# Autodesk Inventor assembly: Vex Pulley 9 mm - 42T
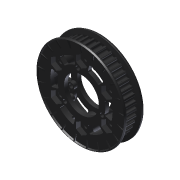
[picture p0: Inventor's stored thumbnail of the model, 180x180]
Saved by Autodesk Inventor 2013 (Build 170138000, 138)
## iProperties
Created: 2013-12-20
Part Number: Vex Pulley 9 mm - 42T
Document SubType Name: Assembly
Designer: Nemo
Author: Nemo
## Documents named in this file (2)
- H:\Nemo\Documents\Robotics\COTS Parts\Pulleys - Vex\Vex Pulley 9 mm - 42T.iam
- H:\Nemo\Documents\Robotics\COTS Parts\Pulleys - Vex\Components\Vex VersaPulley 42T half.ipt
## Components (2 placed, 1 different names)
1. Vex VersaPulley 42T half:1 — Mate:1, Mate:2, Flush:2
2. Vex VersaPulley 42T half:2 — Flush:1, Mate:3, Mate:4
## Relationships (6: Mate 4, Flush 2)
- Flush:1: Vex VersaPulley 42T half:2
- Mate:1: Vex VersaPulley 42T half:1
- Mate:2: Vex VersaPulley 42T half:1
- Mate:3: Vex VersaPulley 42T half:2
- Flush:2: Vex VersaPulley 42T half:1
- Mate:4: Vex VersaPulley 42T half:2
